# Autodesk Inventor assembly: High Strength 84-Tooth Gear, Free Spinning Insert
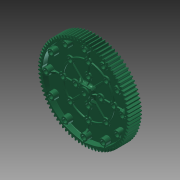
[picture p0: Inventor's stored thumbnail of the model, 180x180]
Saved by Autodesk Inventor 2016 (Build 200138000, 138)
## iProperties
Company: Bots 'n' Stuff
Created: 2014-06-27
Document SubType Name: Assembly
Designer: Jordan Kiesel
Vendor: VEX Robotics, Inc.
Part Number: High Strength 84-Tooth Gear, Free Spinning Insert
Mass: 40.8906 g
Surface Area: 282.55 cm^2
Volume: 28.6952 cm^3
Density: 1.425 g/cm^3
Author: Jordan Kiesel
Title: High Strength 84-Tooth Gear, Square Insert
## Documents named in this file (3)
- C:\Users\Jordan\Documents\Robotics\CAD\2015 BNS CAD Library (beta)\Motion\Spur Gears\High Strength 84-Tooth Gear, Free Spinning Insert.iam
- C:\Users\Jordan\Documents\Robotics\CAD\2015 BNS CAD Library (beta)\Motion\Spur Gears\Reference Parts\High Strength Gears\High Strength 84-Tooth Gear.ipt
- C:\Users\Jordan\Documents\Robotics\CAD\2015 BNS CAD Library (beta)\Motion\Reference Parts\Free Spinning Gear Insert.ipt
## Components (3 placed, 2 different names)
1. High Strength 84-Tooth Gear:1 — Mate:3, Mate:6
2. Free Spinning Gear Insert:1 — Mate:3
3. Free Spinning Gear Insert:2 — Mate:6
## Relationships (6: Mate 6)
- [Mate] (0.0254 mm): High Strength 84-Tooth Gear:1 ↔ Free Spinning Gear Insert:1
- [Mate] (0.0254 mm): High Strength 84-Tooth Gear:1 ↔ Free Spinning Gear Insert:1
- Mate:3: High Strength 84-Tooth Gear:1 ↔ Free Spinning Gear Insert:1
- [Mate] (0.0254 mm): High Strength 84-Tooth Gear:1 ↔ Free Spinning Gear Insert:2
- [Mate] (0.0254 mm): High Strength 84-Tooth Gear:1 ↔ Free Spinning Gear Insert:2
- Mate:6: High Strength 84-Tooth Gear:1 ↔ Free Spinning Gear Insert:2
